# Autodesk Inventor assembly: RRRC_carrier_board
(part 2 of 2)
- C:\!_Dani\!_cloud\OneDrive\!_munka\Revolution\RevvyDemoKit\Structural parts\Demo parts\BrainSofteq\C13_CARRIER_3.iam
- C:\!_Dani\!_cloud\OneDrive\!_munka\Revolution\RevvyDemoKit\Structural parts\Demo parts\BrainSofteq\C12_CARRIER_3.iam
- C:\!_Dani\!_cloud\OneDrive\!_munka\Revolution\RevvyDemoKit\Structural parts\Demo parts\BrainSofteq\C11_CARRIER_3.iam
- C:\!_Dani\!_cloud\OneDrive\!_munka\Revolution\RevvyDemoKit\Structural parts\Demo parts\BrainSofteq\C10_CARRIER_3.iam
- C:\!_Dani\!_cloud\OneDrive\!_munka\Revolution\RevvyDemoKit\Structural parts\Demo parts\BrainSofteq\C9_CARRIER_3.iam
- C:\!_Dani\!_cloud\OneDrive\!_munka\Revolution\RevvyDemoKit\Structural parts\Demo parts\BrainSofteq\C8_CARRIER_3.iam
- C:\!_Dani\!_cloud\OneDrive\!_munka\Revolution\RevvyDemoKit\Structural parts\Demo parts\BrainSofteq\C7_CARRIER_3.iam
- C:\!_Dani\!_cloud\OneDrive\!_munka\Revolution\RevvyDemoKit\Structural parts\Demo parts\BrainSofteq\C6_CARRIER_3.iam
- C:\!_Dani\!_cloud\OneDrive\!_munka\Revolution\RevvyDemoKit\Structural parts\Demo parts\BrainSofteq\C5_CARRIER_3.iam
- C:\!_Dani\!_cloud\OneDrive\!_munka\Revolution\RevvyDemoKit\Structural parts\Demo parts\BrainSofteq\C4_CARRIER_3.iam
- C:\!_Dani\!_cloud\OneDrive\!_munka\Revolution\RevvyDemoKit\Structural parts\Demo parts\BrainSofteq\C3_CARRIER_3.iam
- C:\!_Dani\!_cloud\OneDrive\!_munka\Revolution\RevvyDemoKit\Structural parts\Demo parts\BrainSofteq\C2_CARRIER_3.iam
- C:\!_Dani\!_cloud\OneDrive\!_munka\Revolution\RevvyDemoKit\Structural parts\Demo parts\BrainSofteq\C1_CARRIER_3.iam
## Components (426 placed, 426 different names)
1. Board_CARRIER_3:1 [sub-assembly]
2. D59_CARRIER_3:1 [sub-assembly]
3. D15_CARRIER_3:1 [sub-assembly]
4. C71_CARRIER_3:1 [sub-assembly]
5. D71_CARRIER_3:1 [sub-assembly]
6. D70_CARRIER_3:1 [sub-assembly]
7. D69_CARRIER_3:1 [sub-assembly]
8. D68_CARRIER_3:1 [sub-assembly]
9. D67_CARRIER_3:1 [sub-assembly]
10. D66_CARRIER_3:1 [sub-assembly]
11. D65_CARRIER_3:1 [sub-assembly]
12. D64_CARRIER_3:1 [sub-assembly]
13. D63_CARRIER_3:1 [sub-assembly]
14. D62_CARRIER_3:1 [sub-assembly]
15. D61_CARRIER_3:1 [sub-assembly]
16. D60_CARRIER_3:1 [sub-assembly]
17. D11_CARRIER_3:1 [sub-assembly]
18. R99_CARRIER_3:1 [sub-assembly]
19. D58_CARRIER_3:1 [sub-assembly]
20. D57_CARRIER_3:1 [sub-assembly]
21. D56_CARRIER_3:1 [sub-assembly]
22. R160_CARRIER_3:1 [sub-assembly]
23. R159_CARRIER_3:1 [sub-assembly]
24. R158_CARRIER_3:1 [sub-assembly]
25. Q19_CARRIER_3:1 [sub-assembly]
26. D24_CARRIER_3:1 [sub-assembly]
27. CON1_CARRIER_3:1 [sub-assembly]
28. D54_CARRIER_3:1 [sub-assembly]
29. D55_CARRIER_3:1 [sub-assembly]
30. Q17_CARRIER_3:1 [sub-assembly]
31. Q18_CARRIER_3:1 [sub-assembly]
32. R142_CARRIER_3:1 [sub-assembly]
33. R144_CARRIER_3:1 [sub-assembly]
34. R147_CARRIER_3:1 [sub-assembly]
35. R139_CARRIER_3:1 [sub-assembly]
36. R135_CARRIER_3:1 [sub-assembly]
37. R133_CARRIER_3:1 [sub-assembly]
38. Q16_CARRIER_3:1 [sub-assembly]
39. Q15_CARRIER_3:1 [sub-assembly]
40. D53_CARRIER_3:1 [sub-assembly]
41. D52_CARRIER_3:1 [sub-assembly]
42. D50_CARRIER_3:1 [sub-assembly]
43. D51_CARRIER_3:1 [sub-assembly]
44. Q13_CARRIER_3:1 [sub-assembly]
45. Q14_CARRIER_3:1 [sub-assembly]
46. R126_CARRIER_3:1 [sub-assembly]
47. R127_CARRIER_3:1 [sub-assembly]
48. R132_CARRIER_3:1 [sub-assembly]
49. CON9_CARRIER_2:1 [sub-assembly]
50. C42_CARRIER_3:1 [sub-assembly]
51. C39_CARRIER_3:1 [sub-assembly]
52. C33_CARRIER_3:1 [sub-assembly]
53. C36_CARRIER_3:1 [sub-assembly]
54. C86_CARRIER_3:1 [sub-assembly]
55. C90_CARRIER_3:1 [sub-assembly]
56. D37_CARRIER_3:1 [sub-assembly]
57. D38_CARRIER_3:1 [sub-assembly]
58. D42_CARRIER_3:1 [sub-assembly]
59. D43_CARRIER_3:1 [sub-assembly]
60. U16_CARRIER_3:1 [sub-assembly]
61. R32_CARRIER_3:1 [sub-assembly]
62. R40_CARRIER_3:1 [sub-assembly]
63. R38_CARRIER_3:1 [sub-assembly]
64. R37_CARRIER_3:1 [sub-assembly]
65. R35_CARRIER_3:1 [sub-assembly]
66. R34_CARRIER_3:1 [sub-assembly]
67. R33_CARRIER_3:1 [sub-assembly]
68. R31_CARRIER_3:1 [sub-assembly]
69. Q5_CARRIER_3:1 [sub-assembly]
70. FU8_CARRIER_3:1 [sub-assembly]
71. FU7_CARRIER_3:1 [sub-assembly]
72. D36_CARRIER_3:1 [sub-assembly]
73. D35_CARRIER_3:1 [sub-assembly]
74. D34_CARRIER_3:1 [sub-assembly]
75. C63_CARRIER_3:1 [sub-assembly]
76. C37_CARRIER_3:1 [sub-assembly]
77. C35_CARRIER_3:1 [sub-assembly]
78. C75_CARRIER_3:1 [sub-assembly]
79. C77_CARRIER_3:1 [sub-assembly]
80. C79_CARRIER_3:1 [sub-assembly]
81. C81_CARRIER_3:1 [sub-assembly]
82. D39_CARRIER_3:1 [sub-assembly]
83. D40_CARRIER_3:1 [sub-assembly]
84. D41_CARRIER_3:1 [sub-assembly]
85. FU10_CARRIER_3:1 [sub-assembly]
86. FU9_CARRIER_3:1 [sub-assembly]
87. Q6_CARRIER_3:1 [sub-assembly]
88. R36_CARRIER_3:1 [sub-assembly]
89. R39_CARRIER_3:1 [sub-assembly]
90. R42_CARRIER_3:1 [sub-assembly]
91. R43_CARRIER_3:1 [sub-assembly]
92. R44_CARRIER_3:1 [sub-assembly]
93. R46_CARRIER_3:1 [sub-assembly]
94. R47_CARRIER_3:1 [sub-assembly]
95. R48_CARRIER_3:1 [sub-assembly]
96. C32_CARRIER_3:1 [sub-assembly]
97. C24_CARRIER_3:1 [sub-assembly]
98. C28_CARRIER_3:1 [sub-assembly]
99. C34_CARRIER_3:1 [sub-assembly]
100. C73_CARRIER_3:1 [sub-assembly]
101. D31_CARRIER_3:1 [sub-assembly]
102. D32_CARRIER_3:1 [sub-assembly]
103. D33_CARRIER_3:1 [sub-assembly]
104. U15_CARRIER_3:1 [sub-assembly]
105. U5_CARRIER_3:1 [sub-assembly]
106. R29_CARRIER_3:1 [sub-assembly]
107. R28_CARRIER_3:1 [sub-assembly]
108. R24_CARRIER_3:1 [sub-assembly]
109. R30_CARRIER_3:1 [sub-assembly]
110. Q4_CARRIER_3:1 [sub-assembly]
111. FU6_CARRIER_3:1 [sub-assembly]
112. FU5_CARRIER_3:1 [sub-assembly]
113. D14_CARRIER_3:1 [sub-assembly]
114. D13_CARRIER_3:1 [sub-assembly]
115. D12_CARRIER_3:1 [sub-assembly]
116. C46_CARRIER_3:1 [sub-assembly]
117. C53_CARRIER_3:1 [sub-assembly]
118. C31_CARRIER_3:1 [sub-assembly]
119. C30_CARRIER_3:1 [sub-assembly]
120. C27_CARRIER_3:1 [sub-assembly]
121. C29_CARRIER_3:1 [sub-assembly]
122. R25_CARRIER_3:1 [sub-assembly]
123. R26_CARRIER_3:1 [sub-assembly]
124. R18_CARRIER_3:1 [sub-assembly]
125. R17_CARRIER_3:1 [sub-assembly]
126. C21_CARRIER_3:1 [sub-assembly]
127. C19_CARRIER_3:1 [sub-assembly]
128. C23_CARRIER_3:1 [sub-assembly]
129. C25_CARRIER_3:1 [sub-assembly]
130. C49_CARRIER_3:1 [sub-assembly]
131. C51_CARRIER_3:1 [sub-assembly]
132. D10_CARRIER_3:1 [sub-assembly]
133. D8_CARRIER_3:1 [sub-assembly]
134. D9_CARRIER_3:1 [sub-assembly]
135. FU3_CARRIER_3:1 [sub-assembly]
136. FU4_CARRIER_3:1 [sub-assembly]
137. Q3_CARRIER_3:1 [sub-assembly]
138. R11_CARRIER_3:1 [sub-assembly]
139. R15_CARRIER_3:1 [sub-assembly]
140. R22_CARRIER_3:1 [sub-assembly]
141. R16_CARRIER_3:1 [sub-assembly]
142. R20_CARRIER_3:1 [sub-assembly]
143. R21_CARRIER_3:1 [sub-assembly]
144. U4_CARRIER_3:1 [sub-assembly]
145. R143_CARRIER_3:1 [sub-assembly]
146. C82_CARRIER_3:1 [sub-assembly]
147. C84_CARRIER_3:1 [sub-assembly]
148. C110_CARRIER_3:1 [sub-assembly]
149. C111_CARRIER_3:1 [sub-assembly]
150. C112_CARRIER_3:1 [sub-assembly]
151. D27_CARRIER_3:1 [sub-assembly]
152. D28_CARRIER_3:1 [sub-assembly]
153. FB7_CARRIER_3:1 [sub-assembly]
154. FB16_CARRIER_3:1 [sub-assembly]
155. FU19_CARRIER_3:1 [sub-assembly]
156. FU20_CARRIER_3:1 [sub-assembly]
157. R100_CARRIER_3:1 [sub-assembly]
158. R101_CARRIER_3:1 [sub-assembly]
159. R104_CARRIER_3:1 [sub-assembly]
160. R141_CARRIER_3:1 [sub-assembly]
161. R145_CARRIER_3:1 [sub-assembly]
162. R146_CARRIER_3:1 [sub-assembly]
163. D21_CARRIER_3:1 [sub-assembly]
164. R122_CARRIER_3:1 [sub-assembly]
165. R121_CARRIER_3:1 [sub-assembly]
166. R89_CARRIER_3:1 [sub-assembly]
167. R86_CARRIER_3:1 [sub-assembly]
168. R85_CARRIER_3:1 [sub-assembly]
169. R118_CARRIER_3:1 [sub-assembly]
170. FU14_CARRIER_3:1 [sub-assembly]
171. FU13_CARRIER_3:1 [sub-assembly]
172. FB10_CARRIER_3:1 [sub-assembly]
173. FB4_CARRIER_3:1 [sub-assembly]
174. D19_CARRIER_3:1 [sub-assembly]
175. D18_CARRIER_3:1 [sub-assembly]
176. D17_CARRIER_3:1 [sub-assembly]
177. C101_CARRIER_3:1 [sub-assembly]
178. C99_CARRIER_3:1 [sub-assembly]
179. C100_CARRIER_3:1 [sub-assembly]
180. C72_CARRIER_3:1 [sub-assembly]
181. C70_CARRIER_3:1 [sub-assembly]
182. C74_CARRIER_3:1 [sub-assembly]
183. C76_CARRIER_3:1 [sub-assembly]
184. C102_CARRIER_3:1 [sub-assembly]
185. C103_CARRIER_3:1 [sub-assembly]
186. C105_CARRIER_3:1 [sub-assembly]
187. D20_CARRIER_3:1 [sub-assembly]
188. D22_CARRIER_3:1 [sub-assembly]
189. FB5_CARRIER_3:1 [sub-assembly]
190. FB12_CARRIER_3:1 [sub-assembly]
191. FU15_CARRIER_3:1 [sub-assembly]
192. FU16_CARRIER_3:1 [sub-assembly]
193. R90_CARRIER_3:1 [sub-assembly]
194. R91_CARRIER_3:1 [sub-assembly]
195. R93_CARRIER_3:1 [sub-assembly]
196. R94_CARRIER_3:1 [sub-assembly]
197. R130_CARRIER_3:1 [sub-assembly]
198. R131_CARRIER_3:1 [sub-assembly]
199. CON2_CARRIER_3:1 [sub-assembly]
200. Y1_CARRIER_3:1 [sub-assembly]
201. U30_CARRIER_3:1 [sub-assembly]
202. U29_CARRIER_3:1 [sub-assembly]
203. U13_CARRIER_3:1 [sub-assembly]
204. U27_CARRIER_3:1 [sub-assembly]
205. U12_CARRIER_3:1 [sub-assembly]
206. U25_CARRIER_3:1 [sub-assembly]
207. U11_CARRIER_3:1 [sub-assembly]
208. U10_CARRIER_3:1 [sub-assembly]
209. U20_CARRIER_3:1 [sub-assembly]
210. U18_CARRIER_3:1 [sub-assembly]
211. U3_CARRIER_3:1 [sub-assembly]
212. U14_CARRIER_3:1 [sub-assembly]
213. U9_CARRIER_3:1 [sub-assembly]
214. U8_CARRIER_3:1 [sub-assembly]
215. U7_CARRIER_3:1 [sub-assembly]
216. U6_CARRIER_3:1 [sub-assembly]
217. U2_CARRIER_3:1 [sub-assembly]
218. U1_CARRIER_3:1 [sub-assembly]
219. S1_CARRIER_3:1 [sub-assembly]
220. R157_CARRIER_3:1 [sub-assembly]
221. R156_CARRIER_3:1 [sub-assembly]
222. R155_CARRIER_3:1 [sub-assembly]
223. R154_CARRIER_3:1 [sub-assembly]
224. R153_CARRIER_3:1 [sub-assembly]
225. R152_CARRIER_3:1 [sub-assembly]
226. R151_CARRIER_3:1 [sub-assembly]
227. R150_CARRIER_3:1 [sub-assembly]
228. R149_CARRIER_3:1 [sub-assembly]
229. R148_CARRIER_3:1 [sub-assembly]
230. R140_CARRIER_3:1 [sub-assembly]
231. R138_CARRIER_3:1 [sub-assembly]
232. R137_CARRIER_3:1 [sub-assembly]
233. R136_CARRIER_3:1 [sub-assembly]
234. R134_CARRIER_3:1 [sub-assembly]
235. R129_CARRIER_3:1 [sub-assembly]
236. R128_CARRIER_3:1 [sub-assembly]
237. R125_CARRIER_3:1 [sub-assembly]
238. R124_CARRIER_3:1 [sub-assembly]
239. R123_CARRIER_3:1 [sub-assembly]
240. R120_CARRIER_3:1 [sub-assembly]
241. R119_CARRIER_3:1 [sub-assembly]
242. R117_CARRIER_3:1 [sub-assembly]
243. R116_CARRIER_3:1 [sub-assembly]
244. R115_CARRIER_3:1 [sub-assembly]
245. R112_CARRIER_3:1 [sub-assembly]
246. R111_CARRIER_3:1 [sub-assembly]
247. R110_CARRIER_3:1 [sub-assembly]
248. R109_CARRIER_3:1 [sub-assembly]
249. R108_CARRIER_3:1 [sub-assembly]
250. R107_CARRIER_3:1 [sub-assembly]
251. R106_CARRIER_3:1 [sub-assembly]
252. R105_CARRIER_3:1 [sub-assembly]
253. R98_CARRIER_3:1 [sub-assembly]
254. R96_CARRIER_3:1 [sub-assembly]
255. R95_CARRIER_3:1 [sub-assembly]
256. R87_CARRIER_3:1 [sub-assembly]
257. R84_CARRIER_3:1 [sub-assembly]
258. R83_CARRIER_3:1 [sub-assembly]
259. R82_CARRIER_3:1 [sub-assembly]
260. R81_CARRIER_3:1 [sub-assembly]
261. R80_CARRIER_3:1 [sub-assembly]
262. R79_CARRIER_3:1 [sub-assembly]
263. R78_CARRIER_3:1 [sub-assembly]
264. R77_CARRIER_3:1 [sub-assembly]
265. R76_CARRIER_3:1 [sub-assembly]
266. R75_CARRIER_3:1 [sub-assembly]
267. R74_CARRIER_3:1 [sub-assembly]
268. R73_CARRIER_3:1 [sub-assembly]
269. R72_CARRIER_3:1 [sub-assembly]
270. R71_CARRIER_3:1 [sub-assembly]
271. R70_CARRIER_3:1 [sub-assembly]
272. R69_CARRIER_3:1 [sub-assembly]
273. R68_CARRIER_3:1 [sub-assembly]
274. R67_CARRIER_3:1 [sub-assembly]
275. R66_CARRIER_3:1 [sub-assembly]
276. R65_CARRIER_3:1 [sub-assembly]
277. R64_CARRIER_3:1 [sub-assembly]
278. R63_CARRIER_3:1 [sub-assembly]
279. R62_CARRIER_3:1 [sub-assembly]
280. R61_CARRIER_3:1 [sub-assembly]
281. R60_CARRIER_3:1 [sub-assembly]
282. R59_CARRIER_3:1 [sub-assembly]
283. R58_CARRIER_3:1 [sub-assembly]
284. R57_CARRIER_3:1 [sub-assembly]
285. R56_CARRIER_3:1 [sub-assembly]
286. R55_CARRIER_3:1 [sub-assembly]
287. R54_CARRIER_3:1 [sub-assembly]
288. R53_CARRIER_3:1 [sub-assembly]
289. R52_CARRIER_3:1 [sub-assembly]
290. R51_CARRIER_3:1 [sub-assembly]
291. R50_CARRIER_3:1 [sub-assembly]
292. R49_CARRIER_3:1 [sub-assembly]
293. R45_CARRIER_3:1 [sub-assembly]
294. R41_CARRIER_3:1 [sub-assembly]
295. R27_CARRIER_3:1 [sub-assembly]
296. R23_CARRIER_3:1 [sub-assembly]
297. R19_CARRIER_3:1 [sub-assembly]
298. R14_CARRIER_3:1 [sub-assembly]
299. R13_CARRIER_3:1 [sub-assembly]
300. R12_CARRIER_3:1 [sub-assembly]
301. R10_CARRIER_3:1 [sub-assembly]
302. R9_CARRIER_3:1 [sub-assembly]
303. R8_CARRIER_3:1 [sub-assembly]
304. R7_CARRIER_3:1 [sub-assembly]
305. R6_CARRIER_3:1 [sub-assembly]
306. R5_CARRIER_3:1 [sub-assembly]
307. R4_CARRIER_3:1 [sub-assembly]
308. R3_CARRIER_3:1 [sub-assembly]
309. R2_CARRIER_3:1 [sub-assembly]
310. R1_CARRIER_3:1 [sub-assembly]
311. Q12_CARRIER_3:1 [sub-assembly]
312. Q11_CARRIER_3:1 [sub-assembly]
313. Q10_CARRIER_3:1 [sub-assembly]
314. Q9_CARRIER_3:1 [sub-assembly]
315. Q8_CARRIER_3:1 [sub-assembly]
316. Q7_CARRIER_3:1 [sub-assembly]
317. Q2_CARRIER_3:1 [sub-assembly]
318. Q1_CARRIER_3:1 [sub-assembly]
319. L3_CARRIER_3:1 [sub-assembly]
320. L2_CARRIER_3:1 [sub-assembly]
321. L1_CARRIER_3:1 [sub-assembly]
322. FU18_CARRIER_3:1 [sub-assembly]
323. FU17_CARRIER_3:1 [sub-assembly]
324. FU12_CARRIER_3:1 [sub-assembly]
325. FU11_CARRIER_3:1 [sub-assembly]
326. FU2_CARRIER_3:1 [sub-assembly]
327. FU1_CARRIER_3:1 [sub-assembly]
328. FB14_CARRIER_3:1 [sub-assembly]
329. FB6_CARRIER_3:1 [sub-assembly]
330. FB3_CARRIER_3:1 [sub-assembly]
331. FB2_CARRIER_3:1 [sub-assembly]
332. FB1_CARRIER_3:1 [sub-assembly]
333. D49_CARRIER_3:1 [sub-assembly]
334. D48_CARRIER_3:1 [sub-assembly]
335. D47_CARRIER_3:1 [sub-assembly]
336. D46_CARRIER_3:1 [sub-assembly]
337. D45_CARRIER_3:1 [sub-assembly]
338. D44_CARRIER_3:1 [sub-assembly]
339. D30_CARRIER_3:1 [sub-assembly]
340. D29_CARRIER_3:1 [sub-assembly]
341. D25_CARRIER_3:1 [sub-assembly]
342. D23_CARRIER_3:1 [sub-assembly]
343. D16_CARRIER_3:1 [sub-assembly]
344. D7_CARRIER_3:1 [sub-assembly]
345. D6_CARRIER_3:1 [sub-assembly]
346. D5_CARRIER_3:1 [sub-assembly]
347. D4_CARRIER_3:1 [sub-assembly]
348. D3_CARRIER_3:1 [sub-assembly]
349. D2_CARRIER_3:1 [sub-assembly]
350. D1_CARRIER_3:1 [sub-assembly]
351. CON8_CARRIER_3:1 [sub-assembly]
352. CON7_CARRIER_3:1 [sub-assembly]
353. CON6_CARRIER_3:1 [sub-assembly]
354. CON5_CARRIER_3:1 [sub-assembly]
355. CON4_CARRIER_3:1 [sub-assembly]
356. CON3_CARRIER_3:1 [sub-assembly]
357. C58_CARRIER_3:1 [sub-assembly]
358. C38_CARRIER_3:1 [sub-assembly]
359. C116_CARRIER_3:1 [sub-assembly]
360. C115_CARRIER_3:1 [sub-assembly]
361. C114_CARRIER_3:1 [sub-assembly]
362. C113_CARRIER_3:1 [sub-assembly]
363. C109_CARRIER_3:1 [sub-assembly]
364. C108_CARRIER_3:1 [sub-assembly]
365. C107_CARRIER_3:1 [sub-assembly]
366. C106_CARRIER_3:1 [sub-assembly]
367. C104_CARRIER_3:1 [sub-assembly]
368. C98_CARRIER_3:1 [sub-assembly]
369. C97_CARRIER_3:1 [sub-assembly]
370. C96_CARRIER_3:1 [sub-assembly]
371. C95_CARRIER_3:1 [sub-assembly]
372. C94_CARRIER_3:1 [sub-assembly]
373. C93_CARRIER_3:1 [sub-assembly]
374. C92_CARRIER_3:1 [sub-assembly]
375. C91_CARRIER_3:1 [sub-assembly]
376. C89_CARRIER_3:1 [sub-assembly]
377. C88_CARRIER_3:1 [sub-assembly]
378. C87_CARRIER_3:1 [sub-assembly]
379. C85_CARRIER_3:1 [sub-assembly]
380. C83_CARRIER_3:1 [sub-assembly]
381. C80_CARRIER_3:1 [sub-assembly]
382. C78_CARRIER_3:1 [sub-assembly]
383. C69_CARRIER_3:1 [sub-assembly]
384. C68_CARRIER_3:1 [sub-assembly]
385. C67_CARRIER_3:1 [sub-assembly]
386. C66_CARRIER_3:1 [sub-assembly]
387. C65_CARRIER_3:1 [sub-assembly]
388. C64_CARRIER_3:1 [sub-assembly]
389. C62_CARRIER_3:1 [sub-assembly]
390. C61_CARRIER_3:1 [sub-assembly]
391. C60_CARRIER_3:1 [sub-assembly]
392. C59_CARRIER_3:1 [sub-assembly]
393. C57_CARRIER_3:1 [sub-assembly]
394. C56_CARRIER_3:1 [sub-assembly]
395. C55_CARRIER_3:1 [sub-assembly]
396. C54_CARRIER_3:1 [sub-assembly]
397. C52_CARRIER_3:1 [sub-assembly]
398. C50_CARRIER_3:1 [sub-assembly]
399. C48_CARRIER_3:1 [sub-assembly]
400. C47_CARRIER_3:1 [sub-assembly]
401. C44_CARRIER_3:1 [sub-assembly]
402. C43_CARRIER_3:1 [sub-assembly]
403. C40_CARRIER_3:1 [sub-assembly]
404. C45_CARRIER_3:1 [sub-assembly]
405. C41_CARRIER_3:1 [sub-assembly]
406. C26_CARRIER_3:1 [sub-assembly]
407. C22_CARRIER_3:1 [sub-assembly]
408. C20_CARRIER_3:1 [sub-assembly]
409. C18_CARRIER_3:1 [sub-assembly]
410. C17_CARRIER_3:1 [sub-assembly]
411. C16_CARRIER_3:1 [sub-assembly]
412. C15_CARRIER_3:1 [sub-assembly]
413. C14_CARRIER_3:1 [sub-assembly]
414. C13_CARRIER_3:1 [sub-assembly]
415. C12_CARRIER_3:1 [sub-assembly]
416. C11_CARRIER_3:1 [sub-assembly]
417. C10_CARRIER_3:1 [sub-assembly]
418. C9_CARRIER_3:1 [sub-assembly]
419. C8_CARRIER_3:1 [sub-assembly]
420. C7_CARRIER_3:1 [sub-assembly]
421. C6_CARRIER_3:1 [sub-assembly]
422. C5_CARRIER_3:1 [sub-assembly]
423. C4_CARRIER_3:1 [sub-assembly]
424. C3_CARRIER_3:1 [sub-assembly]
425. C2_CARRIER_3:1 [sub-assembly]
426. C1_CARRIER_3:1 [sub-assembly]
